# Autodesk Inventor assembly: Talp
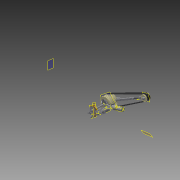
[picture p0: Inventor's stored thumbnail of the model, 180x180]
Saved by Autodesk Inventor 2015 SP1 (Build 190203100, 203)
## iProperties
Created: 2015-02-23
Part Number: Talp
Document SubType Name: Assembly
Designer: laca
Author: laca
## Documents named in this file (20)
- C:\Users\laca\Desktop\RobotMechanika\Talp.iam
- C:\Users\laca\Desktop\RobotMechanika\NagyKerek.ipt
- C:\Users\laca\Desktop\RobotMechanika\NagyTengely.ipt
- C:\Users\laca\Desktop\RobotMechanika\KissKerek.ipt
- C:\Users\laca\Desktop\RobotMechanika\6001 BEARING.iam
- C:\Users\laca\Desktop\RobotMechanika\Alkar.ipt
- C:\Users\laca\Desktop\RobotMechanika\Felkar.ipt
- C:\Users\laca\Desktop\RobotMechanika\KisTenge.ipt
- C:\Users\laca\Desktop\RobotMechanika\SpanoloAnya.ipt
- C:\Users\laca\Desktop\RobotMechanika\Tavolsagtarto.ipt
- C:\Users\laca\Desktop\RobotMechanika\SzenzorCsavar5os.ipt
- C:\Users\laca\Desktop\RobotMechanika\Worm Gear1.ipt
- C:\Users\laca\Desktop\RobotMechanika\Bisztositek.ipt
- C:\Users\laca\Desktop\RobotMechanika\Szij.ipt
- C:\Users\laca\Desktop\RobotMechanika\Bevel Gears2.iam
- C:\Users\laca\Desktop\RobotMechanika\MotorKerekHajtas.iam
- C:\Users\laca\Desktop\RobotMechanika\ISO 7089 - 5 - 140 HV(1).ipt
- C:\Users\laca\Desktop\RobotMechanika\InkrementalisFolia.ipt
- C:\Users\laca\Desktop\RobotMechanika\MotorEsOrsoHajtas.iam
- C:\Users\laca\Desktop\RobotMechanika\JIS B 1181 - M5(1).ipt
## Components (32 placed, 19 different names)
1. NagyKerek:1
2. NagyTengely:1 — Rigid:8, Insert:2, Cylindrical:8
3. 6001 BEARING:1 [sub-assembly]
4. 6001 BEARING:2 [sub-assembly]
5. 6001 BEARING:3 [sub-assembly]
6. 6001 BEARING:4 [sub-assembly]
7. Alkar:1
8. Felkar:1
9. KissKerek:1
10. KisTenge:1
11. SpanoloAnya:1
12. SpanoloAnya:2
13. SpanoloAnya:3 — Insert:2
14. Tavolsagtarto:1
15. SzenzorCsavar5os:1 — Rigid:8, Cylindrical:6, Mate:5, Cylindrical:7
16. Bisztositek:1 — Cylindrical:9, Angle:1, Mate:10
17. Szij:1
18. MotorEsOrsoHajtas:1 [sub-assembly]
19. Bevel Gears:1 [sub-assembly]
20. MotorKerekHajtas:1 [sub-assembly]
21. SpanoloAnya:4 — Insert:14
22. JIS B 1181 finished Class 2 - Metric Class 2 finished M5:1 — Cylindrical:6, Mate:5, Insert:4
23. JIS B 1181 finished Class 2 - Metric Class 2 finished M5:2 — Insert:7
24. ISO 7089 5 - 140 HV:1 — Insert:4, Insert:12, Insert:16
25. ISO 7089 5 - 140 HV:2 — Insert:8, Insert:13, Insert:15
26. ISO 7089 5 - 140 HV:3 — Insert:11, Insert:16
27. ISO 7089 5 - 140 HV:4 — Insert:7, Insert:15
28. JIS B 1181 finished Class 2 - Metric Class 2 finished M5:3 — Insert:11
29. JIS B 1181 finished Class 2 - Metric Class 2 finished M5:4 — Cylindrical:7, Insert:8
30. InkrementalisFolia:1 — Insert:13, Mate:8, Mate:9
31. InkrementalisFolia:2 — Insert:12, Mate:8
32. Worm Gear1:2 — Cylindrical:8, Cylindrical:9, Insert:14, Mate:9, Tangent:1
## Relationships (47: Insert 11, Mate 10, CylindricalJoint 8, WeldJoint 7, RevoluteJoint 7, Flush 1, RelateRotation 1, Angle 1, Tangent 1)
- [WeldJoint]: NagyKerek:1 ↔ 6001 BEARING:1
- [WeldJoint]: NagyKerek:1 ↔ 6001 BEARING:2
- [WeldJoint]: 6001 BEARING:4 ↔ KissKerek:1
- [WeldJoint]: 6001 BEARING:3 ↔ KissKerek:1
- [WeldJoint]: 6001 BEARING:4 ↔ KisTenge:1
- [RevoluteJoint]: 6001 BEARING:3 ↔ SpanoloAnya:2
- [RevoluteJoint]: NagyTengely:1 ↔ 6001 BEARING:2
- [RevoluteJoint]: 6001 BEARING:1 ↔ Tavolsagtarto:1
- Rigid:8 [WeldJoint] (-5 mm): NagyTengely:1 ↔ SzenzorCsavar5os:1
- [WeldJoint]: NagyTengely:1 ↔ Alkar:1
- [CylindricalJoint]: NagyTengely:1 ↔ Bisztositek:1
- [RevoluteJoint]: NagyKerek:1 ↔ Szij:1
- [Mate]: Alkar:1 ↔ Felkar:1
- [Mate]: Alkar:1 ↔ Felkar:1
- [Insert]: Felkar:1 ↔ KisTenge:1
- [RevoluteJoint]: KissKerek:1 ↔ Szij:1
- [Mate]: Alkar:1 ↔ SpanoloAnya:1
- [CylindricalJoint]: Felkar:1 ↔ SpanoloAnya:1
- [Mate]: Alkar:1 ↔ Felkar:1
- [RevoluteJoint]: NagyKerek:1 ↔ Bevel Gears:1
- [RevoluteJoint]: NagyKerek:1 ↔ Bevel Gears:1
- [CylindricalJoint]: Bevel Gears:1 ↔ MotorKerekHajtas:1
- [CylindricalJoint]: Bevel Gears:1 ↔ MotorKerekHajtas:1
- [Flush]: Bevel Gears:1 ↔ MotorKerekHajtas:1
- Insert:2: NagyTengely:1 ↔ SpanoloAnya:3
- Cylindrical:6: SzenzorCsavar5os:1 ↔ JIS B 1181 finished Class 2 - Metric Class 2 finished M5:1
- Mate:5: SzenzorCsavar5os:1 ↔ JIS B 1181 finished Class 2 - Metric Class 2 finished M5:1
- Insert:4: JIS B 1181 finished Class 2 - Metric Class 2 finished M5:1 ↔ ISO 7089 5 - 140 HV:1
- Insert:7: JIS B 1181 finished Class 2 - Metric Class 2 finished M5:2 ↔ ISO 7089 5 - 140 HV:4
- Cylindrical:7: SzenzorCsavar5os:1 ↔ JIS B 1181 finished Class 2 - Metric Class 2 finished M5:4
- Insert:8: ISO 7089 5 - 140 HV:2 ↔ JIS B 1181 finished Class 2 - Metric Class 2 finished M5:4
- Insert:11: ISO 7089 5 - 140 HV:3 ↔ JIS B 1181 finished Class 2 - Metric Class 2 finished M5:3
- Insert:12: ISO 7089 5 - 140 HV:1 ↔ InkrementalisFolia:2
- Insert:13: ISO 7089 5 - 140 HV:2 ↔ InkrementalisFolia:1
- [Mate]: MotorEsOrsoHajtas:1 ↔ Worm Gear1:2
- [Mate] (41.004 mm): MotorEsOrsoHajtas:1 ↔ Worm Gear1:2
- [RelateRotation] (66 ul): MotorEsOrsoHajtas:1 ↔ Worm Gear1:2
- Cylindrical:8: NagyTengely:1 ↔ Worm Gear1:2
- Cylindrical:9: Bisztositek:1 ↔ Worm Gear1:2
- Insert:14: SpanoloAnya:4 ↔ Worm Gear1:2
- Mate:8 (15 mm): InkrementalisFolia:1 ↔ InkrementalisFolia:2
- Insert:15: ISO 7089 5 - 140 HV:2 ↔ ISO 7089 5 - 140 HV:4
- Insert:16: ISO 7089 5 - 140 HV:1 ↔ ISO 7089 5 - 140 HV:3
- Mate:9: InkrementalisFolia:1 ↔ Worm Gear1:2
- Angle:1 (0 deg): Bisztositek:1
- Tangent:1: Worm Gear1:2
- Mate:10: Bisztositek:1
## Named parameters: d31_d40 = 0 mm, d32_d41 = -62.564717 deg, d37_d38 = 0 mm, d38_d39 = 133.38057 deg
